# Autodesk Inventor assembly: Assembly_HoliSheet_v6
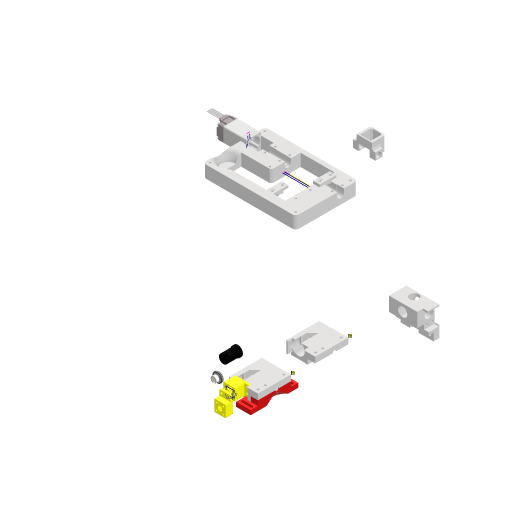
[picture p0: Inventor's stored thumbnail of the model, 512x512]
Saved by Autodesk Inventor 2024.1 (Build 281209000, 209)
## iProperties
Created: 2023-01-07
Part Number: Assembly_HoliSheet_v6
Document SubType Name: Assembly
Designer: diederichbenedict
Author: diederichbenedict
## Documents named in this file (10)
- C:\Users\diederichbenedict\Dropbox\Dokumente\Promotion\PROJECTS\HoLiSheet\INVENTOR\Assembly_HoliSheet_v6.iam
- C:\Users\diederichbenedict\Dropbox\Dokumente\Promotion\PROJECTS\HoLiSheet\INVENTOR\Assemlby_Scanner_v1.iam
- C:\Users\diederichbenedict\Dropbox\Dokumente\Promotion\PROJECTS\HoLiSheet\INVENTOR\11_Wellplatespacer.ipt
- C:\Users\diederichbenedict\Dropbox\Dokumente\Promotion\PROJECTS\HoLiSheet\INVENTOR\00_microscope_turret.ipt
- C:\Users\diederichbenedict\Dropbox\Dokumente\Promotion\PROJECTS\HoLiSheet\INVENTOR\00_NEMA8.ipt
- C:\Users\diederichbenedict\Dropbox\Dokumente\Promotion\PROJECTS\HoLiSheet\INVENTOR\10_Wellplate_base_v6.ipt
- C:\Users\diederichbenedict\Dropbox\Dokumente\Promotion\PROJECTS\HoLiSheet\INVENTOR\Holisheet_tubeclamp.ipt
- C:\Users\diederichbenedict\Dropbox\Dokumente\Promotion\PROJECTS\HoLiSheet\INVENTOR\11_Wellplatespacer_magnetic.ipt
- C:\Users\diederichbenedict\Dropbox\Dokumente\Promotion\PROJECTS\HoLiSheet\INVENTOR\Assemlby_lightsheet_generator_passive_v2.iam
- C:\Users\diederichbenedict\Dropbox\Dokumente\Promotion\PROJECTS\HoLiSheet\INVENTOR\HolisheetCageSampleWater.ipt
## Components (11 placed, 9 different names)
1. 10_Wellplate_base_v6:1 — Passend:2, Winkel:1, Einfügen:1, Winkel:2, Fluchtend:1, Fluchtend:2, Einfügen:2, Winkel:3, Fluchtend:8, Fluchtend:9, Fluchtend:10, Fluchtend:11, Fluchtend:12
2. Assemlby_Scanner_v1:1 [sub-assembly] — Passend:2, Winkel:1, Fluchtend:1, Fluchtend:2
3. 11_Wellplatespacer:1 — Einfügen:1, Winkel:2
4. 00_microscope_turret:1
5. 00_NEMA8:1 — Einfügen:2, Winkel:3
6. Holisheet_tubeclamp:1 — Fluchtend:8, Fluchtend:9, Fluchtend:10
7. Holisheet_tubeclamp:2
8. 11_Wellplatespacer_magnetic:1
9. Assemlby_lightsheet_generator_passive_v2:1 [sub-assembly]
10. HolisheetCageSampleWater:1 — Fluchtend:11, Fluchtend:12
11. Holisheet_tubeclamp:3
## Relationships (13: Flush 7, Angle 3, Insert 2, Mate 1)
- Passend:2 [Mate] (1.4 mm): 10_Wellplate_base_v6:1 ↔ Assemlby_Scanner_v1:1
- Winkel:1 [Angle] (0 deg): 10_Wellplate_base_v6:1 ↔ Assemlby_Scanner_v1:1
- Einfügen:1 [Insert]: 10_Wellplate_base_v6:1 ↔ 11_Wellplatespacer:1
- Winkel:2 [Angle] (180 deg): 10_Wellplate_base_v6:1 ↔ 11_Wellplatespacer:1
- Fluchtend:1 [Flush]: 10_Wellplate_base_v6:1 ↔ Assemlby_Scanner_v1:1
- Fluchtend:2 [Flush]: 10_Wellplate_base_v6:1 ↔ Assemlby_Scanner_v1:1
- Einfügen:2 [Insert]: 10_Wellplate_base_v6:1 ↔ 00_NEMA8:1
- Winkel:3 [Angle] (180 deg): 10_Wellplate_base_v6:1 ↔ 00_NEMA8:1
- Fluchtend:8 [Flush]: 10_Wellplate_base_v6:1 ↔ Holisheet_tubeclamp:1
- Fluchtend:9 [Flush]: 10_Wellplate_base_v6:1 ↔ Holisheet_tubeclamp:1
- Fluchtend:10 [Flush]: 10_Wellplate_base_v6:1 ↔ Holisheet_tubeclamp:1
- Fluchtend:11 [Flush]: 10_Wellplate_base_v6:1 ↔ HolisheetCageSampleWater:1
- Fluchtend:12 [Flush]: 10_Wellplate_base_v6:1 ↔ HolisheetCageSampleWater:1
